# Autodesk Inventor assembly: Omni Roller 4 in
Saved by Autodesk Inventor 2013 (Build 170138000, 138)
## iProperties
Created: 2013-01-03
Part Number: Omni Roller 4 in
Document SubType Name: Assembly
Designer: Nemo
Author: Nemo
## Documents named in this file (4)
- H:\Nemo\Documents\Robotics\VexPro\Omni Wheel\Components\Omni Roller 4 in.iam
- H:\Nemo\Documents\Robotics\VexPro\Omni Wheel\Components\Omni Roller 4 in.ipt
- H:\Nemo\Documents\Robotics\VexPro\Omni Wheel\Components\Omni Roller Bearing.ipt
- H:\Nemo\Documents\Robotics\VexPro\Omni Wheel\Components\Omni Roller Shaft 4 in.ipt
## Components (4 placed, 3 different names)
1. Omni Roller 4 in:1
2. Omni Roller Bearing:1
3. Omni Roller Shaft 4 in:1
4. Omni Roller Bearing:2
## Relationships (4: Insert 2, Mate 2)
- [Insert]: Omni Roller 4 in:1 ↔ Omni Roller Bearing:1
- [Insert]: Omni Roller 4 in:1 ↔ Omni Roller Bearing:2
- [Mate]: Omni Roller 4 in:1 ↔ Omni Roller Shaft 4 in:1
- [Mate]: Omni Roller 4 in:1 ↔ Omni Roller Shaft 4 in:1
